# Autodesk Inventor assembly: uMule-UDaR
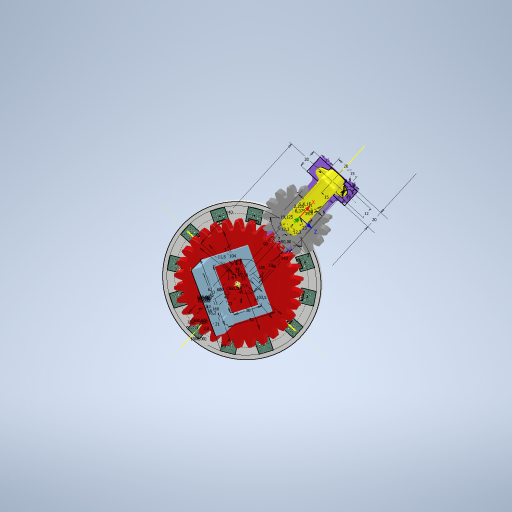
[picture p0: Inventor's stored thumbnail of the model, 512x512]
Saved by Autodesk Inventor 2024.2 (Build 282272000, 272)
## iProperties
Created: 2024-10-14
Part Number: uMule-UDaR
Document SubType Name: Assembly
Designer: owozn
Author: owozn
## Documents named in this file (10)
- C:\Users\owozn\Documents\Semestr 7\Inżynierka\Modele 3D\uMule-UDaR.iam
- C:\Users\owozn\Downloads\Part Studio 1 - Spur gear (15 teeth) (2)\Part Studio 1 - Spur gear (15 teeth) (2).ipt
- C:\Users\owozn\Documents\Semestr 7\Inżynierka\Modele 3D\Slip ring\SlipRing_with_Flange_22mm\SlipRing_with_Flange_22mm.ipt
- C:\Users\owozn\Documents\Semestr 7\Inżynierka\Modele 3D\uMule-UDaR-main_gear.ipt
- C:\Users\owozn\Documents\Semestr 7\Inżynierka\Modele 3D\uMule-UDaR-sensor.ipt
- C:\Users\owozn\Documents\Semestr 7\Inżynierka\Modele 3D\uMule_uchwyt-sens.ipt
- C:\Users\owozn\Documents\Semestr 7\Inżynierka\Modele 3D\tower-pro-mg90s-micro-servo-2.snapshot.3\Tower Pro MG90S Micro servo\Tower Pro MG90S Micro servo.ipt
- C:\Users\owozn\Documents\Semestr 7\Inżynierka\Modele 3D\uMule-uchwyt_servo.ipt
- C:\Users\owozn\Documents\Semestr 7\Inżynierka\Modele 3D\uMule-podstawka_czujnikiIR.ipt
- C:\Users\owozn\Documents\Semestr 7\Inżynierka\Modele 3D\uMule-IR\uMule-IR.ipt
## Components (19 placed, 9 different names)
1. Part Studio 1 - Spur gear (15 teeth) (2):1 — Zestawiające:1, Równoległe:1, Zestawiające:11, Zestawiające:12, Zestawiające:17
2. SlipRing_with_Flange_22mm:1 — Zestawiające:3, Zestawiające:7, Zestawiające:9, Zestawiające:14, Zestawiające:15
3. uMule-UDaR-main_gear:1 — Zestawiające:1, Zestawiające:3, Równoległe:1, Zestawiające:4, Zestawiające:5, Zestawiające:6, Zestawiające:15
4. uMule-UDaR-sensor:1 — Zestawiające:4, Zestawiające:5, Zestawiające:6
5. uMule_uchwyt-sens:1 — Zestawiające:7, Zestawiające:9, Zestawiające:13, Zestawiające:14, Równoległe:2, Zestawiające:18, Zestawiające:19, Zestawiające:20, Równoległe:12
6. Tower Pro MG90S Micro servo:1 — Zestawiające:11, Zestawiające:12, Zestawiające:13
7. uMule-uchwyt_servo:1 — Równoległe:2, Zestawiające:17, Zestawiające:18
8. uMule-podstawka_czujnikiIR:1 — Zestawiające:19, Zestawiające:20, Zestawiające:21, Równoległe:12, Zestawiające:22, Zestawiające:23, Zestawiające:24, Zestawiające:25, Zestawiające:26, Zestawiające:27, Zestawiające:28, Zestawiające:29, Zestawiające:30, Zestawiające:31, Zestawiające:32, Zestawiające:33, Zestawiające:34, Zestawiające:35, Zestawiające:36, Zestawiające:37, Zestawiające:38, Zestawiające:39, Zestawiające:40, Zestawiające:41, Zestawiające:42, Zestawiające:43
9. uMule-IR:1 — Równoległe:8, Równoległe:10, Zestawiające:30, Zestawiające:31
10. uMule-IR:2 — Równoległe:5, Równoległe:6, Równoległe:8, Równoległe:9, Zestawiające:38, Zestawiające:39
11. uMule-IR:3 — Równoległe:4, Równoległe:5, Zestawiające:32, Zestawiające:33
12. uMule-IR:4 — Równoległe:6, Równoległe:7, Równoległe:13, Zestawiające:40, Zestawiające:41
13. uMule-IR:5 — Równoległe:11, Zestawiające:36, Zestawiające:37
14. uMule-IR:6 — Równoległe:10, Równoległe:11, Zestawiające:34, Zestawiające:35
15. uMule-IR:7 — Równoległe:9, Zestawiające:28, Zestawiające:29
16. uMule-IR:8 — Równoległe:3, Równoległe:4, Zestawiające:21, Zestawiające:22, Zestawiające:23
17. uMule-IR:9 — Równoległe:3, Zestawiające:24, Zestawiające:25
18. uMule-IR:10 — Równoległe:7, Zestawiające:42, Zestawiające:43
19. uMule-IR:11 — Równoległe:13, Zestawiające:26, Zestawiające:27
## Relationships (52: Mate 39, Flush 13)
- Zestawiające:1 [Mate] (90 mm): Part Studio 1 - Spur gear (15 teeth) (2):1 ↔ uMule-UDaR-main_gear:1
- Zestawiające:3 [Mate] (2 mm): SlipRing_with_Flange_22mm:1 ↔ uMule-UDaR-main_gear:1
- Równoległe:1 [Flush]: Part Studio 1 - Spur gear (15 teeth) (2):1 ↔ uMule-UDaR-main_gear:1
- Zestawiające:4 [Mate]: uMule-UDaR-main_gear:1 ↔ uMule-UDaR-sensor:1
- Zestawiające:5 [Mate]: uMule-UDaR-main_gear:1 ↔ uMule-UDaR-sensor:1
- Zestawiające:6 [Mate]: uMule-UDaR-main_gear:1 ↔ uMule-UDaR-sensor:1
- Zestawiające:7 [Mate]: SlipRing_with_Flange_22mm:1 ↔ uMule_uchwyt-sens:1
- Zestawiające:9 [Mate]: SlipRing_with_Flange_22mm:1 ↔ uMule_uchwyt-sens:1
- Zestawiające:11 [Mate]: Part Studio 1 - Spur gear (15 teeth) (2):1 ↔ Tower Pro MG90S Micro servo:1
- Zestawiające:12 [Mate]: Part Studio 1 - Spur gear (15 teeth) (2):1 ↔ Tower Pro MG90S Micro servo:1
- Zestawiające:13 [Mate]: uMule_uchwyt-sens:1 ↔ Tower Pro MG90S Micro servo:1
- Zestawiające:14 [Mate]: SlipRing_with_Flange_22mm:1 ↔ uMule_uchwyt-sens:1
- Zestawiające:15 [Mate]: SlipRing_with_Flange_22mm:1 ↔ uMule-UDaR-main_gear:1
- Równoległe:2 [Flush]: uMule_uchwyt-sens:1 ↔ uMule-uchwyt_servo:1
- Zestawiające:17 [Mate]: Part Studio 1 - Spur gear (15 teeth) (2):1 ↔ uMule-uchwyt_servo:1
- Zestawiające:18 [Mate]: uMule_uchwyt-sens:1 ↔ uMule-uchwyt_servo:1
- Zestawiające:19 [Mate]: uMule_uchwyt-sens:1 ↔ uMule-podstawka_czujnikiIR:1
- Zestawiające:20 [Mate] (0.5 mm): uMule_uchwyt-sens:1 ↔ uMule-podstawka_czujnikiIR:1
- Równoległe:3 [Flush]: uMule-IR:8 ↔ uMule-IR:9
- Równoległe:4 [Flush]: uMule-IR:3 ↔ uMule-IR:8
- Równoległe:5 [Flush]: uMule-IR:2 ↔ uMule-IR:3
- Równoległe:6 [Flush]: uMule-IR:2 ↔ uMule-IR:4
- Równoległe:7 [Flush]: uMule-IR:4 ↔ uMule-IR:10
- Równoległe:8 [Flush]: uMule-IR:1 ↔ uMule-IR:2
- Równoległe:9 [Flush]: uMule-IR:2 ↔ uMule-IR:7
- Równoległe:10 [Flush]: uMule-IR:1 ↔ uMule-IR:6
- Równoległe:11 [Flush]: uMule-IR:5 ↔ uMule-IR:6
- Zestawiające:21 [Mate]: uMule-podstawka_czujnikiIR:1 ↔ uMule-IR:8
- Równoległe:12 [Flush]: uMule_uchwyt-sens:1 ↔ uMule-podstawka_czujnikiIR:1
- Zestawiające:22 [Mate]: uMule-podstawka_czujnikiIR:1 ↔ uMule-IR:8
- Zestawiające:23 [Mate]: uMule-podstawka_czujnikiIR:1 ↔ uMule-IR:8
- Zestawiające:24 [Mate]: uMule-podstawka_czujnikiIR:1 ↔ uMule-IR:9
- Zestawiające:25 [Mate]: uMule-podstawka_czujnikiIR:1 ↔ uMule-IR:9
- Równoległe:13 [Flush]: uMule-IR:4 ↔ uMule-IR:11
- Zestawiające:26 [Mate]: uMule-podstawka_czujnikiIR:1 ↔ uMule-IR:11
- Zestawiające:27 [Mate]: uMule-podstawka_czujnikiIR:1 ↔ uMule-IR:11
- Zestawiające:28 [Mate]: uMule-podstawka_czujnikiIR:1 ↔ uMule-IR:7
- Zestawiające:29 [Mate]: uMule-podstawka_czujnikiIR:1 ↔ uMule-IR:7
- Zestawiające:30 [Mate]: uMule-podstawka_czujnikiIR:1 ↔ uMule-IR:1
- Zestawiające:31 [Mate]: uMule-podstawka_czujnikiIR:1 ↔ uMule-IR:1
- Zestawiające:32 [Mate]: uMule-podstawka_czujnikiIR:1 ↔ uMule-IR:3
- Zestawiające:33 [Mate]: uMule-podstawka_czujnikiIR:1 ↔ uMule-IR:3
- Zestawiające:34 [Mate]: uMule-podstawka_czujnikiIR:1 ↔ uMule-IR:6
- Zestawiające:35 [Mate]: uMule-podstawka_czujnikiIR:1 ↔ uMule-IR:6
- Zestawiające:36 [Mate]: uMule-podstawka_czujnikiIR:1 ↔ uMule-IR:5
- Zestawiające:37 [Mate]: uMule-podstawka_czujnikiIR:1 ↔ uMule-IR:5
- Zestawiające:38 [Mate]: uMule-podstawka_czujnikiIR:1 ↔ uMule-IR:2
- Zestawiające:39 [Mate]: uMule-podstawka_czujnikiIR:1 ↔ uMule-IR:2
- Zestawiające:40 [Mate]: uMule-podstawka_czujnikiIR:1 ↔ uMule-IR:4
- Zestawiające:41 [Mate]: uMule-podstawka_czujnikiIR:1 ↔ uMule-IR:4
- Zestawiające:42 [Mate]: uMule-podstawka_czujnikiIR:1 ↔ uMule-IR:10
- Zestawiające:43 [Mate]: uMule-podstawka_czujnikiIR:1 ↔ uMule-IR:10
## Named parameters: Finish1_Area = 68.2082
note: some values were not read from the file. Shown as the stored number, unit unknown: "Finish1_Area".
